# Autodesk Inventor assembly: drivebase V2
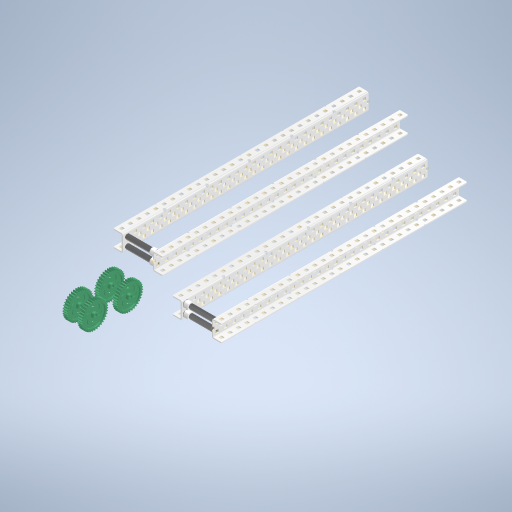
[picture p0: Inventor's stored thumbnail of the model, 512x512]
Saved by Autodesk Inventor 2023 (Build 270158000, 158)
## iProperties
Created: 2023-11-07
Part Number: drivebase V2
Document SubType Name: Assembly
Designer: Robodox
Author: Robodox
## Documents named in this file (9)
- C:\Users\Robodox\Documents\GitHub\2023-599Z\BBotCAD\drivebase V2.iam
- C:\Users\Robodox\Documents\GitHub\2023-599Z\BBotCAD\VEX-CAD-Inventor-1.4.0\Structure\Standoff.ipt
- C:\Users\Robodox\Documents\GitHub\2023-599Z\BBotCAD\VEX-CAD-Inventor-1.4.0\Structure\C Channel\Aluminum 1x2x1\Alu C 1x2x1x29.ipt
- C:\Users\Robodox\Documents\GitHub\2023-599Z\BBotCAD\VEX-CAD-Inventor-1.4.0\Motion\Spacers\Spacer Nylon .313 OD\NSpacer .313 OD x .250.ipt
- C:\Users\Robodox\Documents\GitHub\2023-599Z\BBotCAD\VEX-CAD-Inventor-1.4.0\Motion\Spacers\Spacer Nylon .313 OD.ipt
- C:\Users\Robodox\Documents\GitHub\2023-599Z\BBotCAD\VEX-CAD-Inventor-1.4.0\Motion\Spacers\Washer Steel\SWasher .375 OD x .031250.ipt
- C:\Users\Robodox\Documents\GitHub\2023-599Z\BBotCAD\VEX-CAD-Inventor-1.4.0\Motion\Spacers\Washer Steel.ipt
- C:\Users\Robodox\Documents\GitHub\2023-599Z\BBotCAD\VEX-CAD-Inventor-1.4.0\Structure\Standoff\Standoff 1.50.ipt
- C:\Users\Robodox\Documents\GitHub\2023-599Z\BBotCAD\VEX-CAD-Inventor-1.4.0\Motion\Gears\LS 36T Gear.ipt
## Components (20 placed, 5 different names)
1. Alu C 1x2x1x29:1 — Mate:14
2. Alu C 1x2x1x29:2 — Mate:1, Mate:4
3. Alu C 1x2x1x29:3 — Mate:7
4. Alu C 1x2x1x29:4 — Mate:8, Mate:9
5. SWasher .375 OD x .031250:1 — Mate:9, Mate:11
6. SWasher .375 OD x .031250:2 — Mate:1, Mate:2
7. SWasher .375 OD x .031250:3 — Mate:8, Mate:10
8. SWasher .375 OD x .031250:4 — Mate:4, Mate:5
9. NSpacer .313 OD x .250:1 — Mate:2, Mate:3
10. NSpacer .313 OD x .250:2 — Mate:11, Mate:13
11. NSpacer .313 OD x .250:3 — Mate:5, Mate:6
12. NSpacer .313 OD x .250:4 — Mate:10, Mate:12
13. Standoff 1.50:1 — Mate:6
14. Standoff 1.50:2 — Mate:12, Mate:14
15. Standoff 1.50:3 — Mate:3, Mate:7
16. Standoff 1.50:4 — Mate:13
17. LS 36T Gear:1
18. LS 36T Gear:2
19. LS 36T Gear:3
20. LS 36T Gear:4
## Relationships (14: Mate 14)
- Mate:1: Alu C 1x2x1x29:2 ↔ SWasher .375 OD x .031250:2
- Mate:2: SWasher .375 OD x .031250:2 ↔ NSpacer .313 OD x .250:1
- Mate:3: NSpacer .313 OD x .250:1 ↔ Standoff 1.50:3
- Mate:4: Alu C 1x2x1x29:2 ↔ SWasher .375 OD x .031250:4
- Mate:5: SWasher .375 OD x .031250:4 ↔ NSpacer .313 OD x .250:3
- Mate:6: NSpacer .313 OD x .250:3 ↔ Standoff 1.50:1
- Mate:7: Alu C 1x2x1x29:3 ↔ Standoff 1.50:3
- Mate:8: Alu C 1x2x1x29:4 ↔ SWasher .375 OD x .031250:3
- Mate:9: Alu C 1x2x1x29:4 ↔ SWasher .375 OD x .031250:1
- Mate:10: SWasher .375 OD x .031250:3 ↔ NSpacer .313 OD x .250:4
- Mate:11: SWasher .375 OD x .031250:1 ↔ NSpacer .313 OD x .250:2
- Mate:12: NSpacer .313 OD x .250:4 ↔ Standoff 1.50:2
- Mate:13: NSpacer .313 OD x .250:2 ↔ Standoff 1.50:4
- Mate:14: Alu C 1x2x1x29:1 ↔ Standoff 1.50:2
